# Autodesk Inventor assembly: Cube 1x1 V5 (USB Laser)
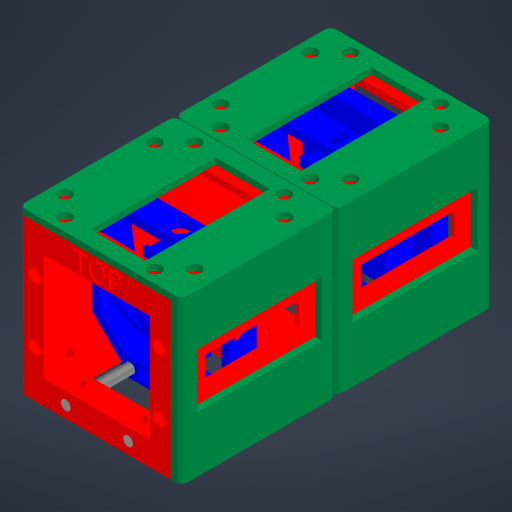
[picture p0: Inventor's stored thumbnail of the model, 512x512]
Saved by Autodesk Inventor 2023.4 (Build 274418000, 418)
## iProperties
Created: 2022-08-13
Part Number: Cube 1x1 V5 (USB Laser)
Document SubType Name: Assembly
Designer: xSibe
Author: xSibe
## Documents named in this file (6)
- C:\.Laptop\.Work\Projects\Project Protocube\Protocube\CAD, STL, OBJ Files\1 CAD\Laser\Cube 1x1 V5 (USB Laser).iam
- C:\.Laptop\.Work\Projects\Project Protocube\Protocube\CAD, STL, OBJ Files\1 CAD\Accessories\Mounting Bar.ipt
- C:\.Laptop\.Work\Projects\Project Protocube\Protocube\CAD, STL, OBJ Files\1 CAD\Filter\Filter Mount (SM1).ipt
- C:\.Laptop\.Work\Projects\Project Protocube\Protocube\CAD, STL, OBJ Files\1 CAD\Laser\Laser Holder (USB Laser).ipt
- C:\.Laptop\.Work\Projects\Project Protocube\Protocube\CAD, STL, OBJ Files\1 CAD\Cubes\Cube 1x1 V5 Laser.iam
- C:\.Laptop\.Work\Projects\Project Protocube\Protocube\CAD, STL, OBJ Files\1 CAD\Covers\Outer Cover Open.ipt
## Components (9 placed, 5 different names)
1. Filter Mount (SM1):1 — Mate:4, Mate:5, Mate:11
2. Cube 1x1 V5 Laser:1 [sub-assembly] — Mate:8, Mate:9, Mate:10
3. Mounting Bar:1 — Flush:1, Mate:4, Mate:5, Mate:6, Mate:7
4. Outer Cover Open:1 — Mate:8, Mate:9, Mate:10
5. Laser Holder (USB Laser):1 — Mate:6, Mate:7, Flush:2
6. Cube 1x1 V5 Laser:2 [sub-assembly] — Mate:11
7. Mounting Bar:2
8. Outer Cover Open:2
9. Laser Holder (USB Laser):2
## Component patterns: (2 elements, first: Cube 1x1 V5 Laser:1 + Mounting Bar:1 + Outer Cover Open:1 + Laser Holder (USB Laser):1)
## Relationships (10: Mate 8, Flush 2)
- Flush:1: Mounting Bar:1
- Mate:4: Filter Mount (SM1):1 ↔ Mounting Bar:1
- Mate:5: Filter Mount (SM1):1 ↔ Mounting Bar:1
- Mate:6: Mounting Bar:1 ↔ Laser Holder (USB Laser):1
- Mate:7: Mounting Bar:1 ↔ Laser Holder (USB Laser):1
- Flush:2: Laser Holder (USB Laser):1
- Mate:8: Cube 1x1 V5 Laser:1 ↔ Outer Cover Open:1
- Mate:9: Cube 1x1 V5 Laser:1 ↔ Outer Cover Open:1
- Mate:10: Cube 1x1 V5 Laser:1 ↔ Outer Cover Open:1
- Mate:11: Filter Mount (SM1):1 ↔ Cube 1x1 V5 Laser:2
